# Autodesk Inventor assembly: Assembly_all
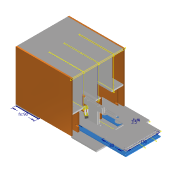
[picture p0: Inventor's stored thumbnail of the model, 180x180]
Saved by Autodesk Inventor 2020 (Build 240168000, 168)
## iProperties
Created: 2021-05-08
Part Number: Assembly_all
Document SubType Name: Assembly
Designer: Hsu Daniel
Author: Hsu Daniel
## Documents named in this file (14)
- D:\Daniel\NTU\makeNTU2021\大改\Assembly_all.iam
- D:\Daniel\NTU\makeNTU2021\大改\lr_heater_assemble.iam
- D:\Daniel\NTU\makeNTU2021\大改\mid_heater_assemble.iam
- D:\Daniel\NTU\makeNTU2021\大改\heater_top.ipt
- D:\Daniel\NTU\makeNTU2021\大改\side_wall.ipt
- D:\Daniel\NTU\makeNTU2021\大改\bottom_inner_wall.ipt
- D:\Daniel\NTU\makeNTU2021\大改\deepest_layer.ipt
- D:\Daniel\NTU\makeNTU2021\大改\Ushape_bottom.ipt
- D:\Daniel\NTU\makeNTU2021\大改\Ushape_top.ipt
- D:\Daniel\NTU\makeNTU2021\大改\Stepper 28BYJ48.ipt
- D:\Daniel\NTU\makeNTU2021\大改\motor_connect.iam
- D:\Daniel\NTU\makeNTU2021\大改\rotate_support.ipt
- D:\Daniel\NTU\makeNTU2021\大改\wire_bottom.ipt
- D:\Daniel\NTU\makeNTU2021\大改\lr_heater_assembleL.iam
## Components (18 placed, 13 different names)
1. lr_heater_assemble:1 [sub-assembly] — Flush:2, Flush:4, Mate:5, Flush:31
2. mid_heater_assemble:1 [sub-assembly] — Flush:2, Flush:4, Mate:1, Mate:2, Mate:3, Mate:9, Mate:10, Flush:28, Flush:29, Flush:32
3. heater_top:1 — Mate:1, Mate:2, Mate:3, Mate:5, Mate:6, Mate:7, Flush:7, Flush:8, Flush:27, Flush:33, Flush:34
4. side_wall:1 — Mate:6, Flush:7, Flush:18, Flush:33
5. side_wall:2 — Mate:7, Flush:8, Flush:26, Flush:34
6. bottom_inner_wall:1 — Flush:11, Flush:14, Flush:31, Mate:25, Mate:26, Mate:27, Mate:28
7. bottom_inner_wall:2 — Flush:10, Flush:11, Flush:13, Flush:14, Mate:12, Mate:24, Mate:29
8. bottom_inner_wall:3 — Flush:9, Flush:10, Flush:15, Mate:9
9. bottom_inner_wall:4 — Flush:9, Flush:13, Flush:15, Mate:10
10. deepest_layer:1 — Flush:18, Mate:12, Mate:14, Flush:26, Mate:24, Mate:25
11. Ushape_bottom:1 — Mate:14, Flush:20, Flush:21, Mate:16, Flush:32, Cylindrical:1
12. Ushape_top:1 — Flush:20, Flush:21, Mate:16, Flush:25, Mate:18, Mate:19, Mate:20, Insert:1
13. Stepper 28BYJ48:1 — Mate:17, Cylindrical:1, Insert:1, Cylindrical:2
14. motor_connect:1 [sub-assembly] — Mate:17, Cylindrical:2
15. rotate_support:1 — Flush:22, Flush:23, Flush:24, Mate:19, Mate:20
16. rotate_support:2 — Flush:22, Flush:23, Flush:24, Flush:25, Mate:18
17. lr_heater_assembleL:1 [sub-assembly] — Flush:27, Flush:28, Flush:29, Mate:29
18. wire_bottom:1 — Mate:26, Mate:27, Mate:28
## Relationships (49: Flush 25, Mate 21, CylindricalJoint 2, Insert 1)
- Flush:2: lr_heater_assemble:1 ↔ mid_heater_assemble:1
- Flush:4: lr_heater_assemble:1 ↔ mid_heater_assemble:1
- Mate:1: mid_heater_assemble:1 ↔ heater_top:1
- Mate:2: mid_heater_assemble:1 ↔ heater_top:1
- Mate:3: mid_heater_assemble:1 ↔ heater_top:1
- Mate:5: lr_heater_assemble:1 ↔ heater_top:1
- Mate:6: heater_top:1 ↔ side_wall:1
- Mate:7: heater_top:1 ↔ side_wall:2
- Flush:7: heater_top:1 ↔ side_wall:1
- Flush:8: heater_top:1 ↔ side_wall:2
- Flush:9: bottom_inner_wall:3 ↔ bottom_inner_wall:4
- Flush:10: bottom_inner_wall:2 ↔ bottom_inner_wall:3
- Flush:11: bottom_inner_wall:1 ↔ bottom_inner_wall:2
- Flush:13: bottom_inner_wall:2 ↔ bottom_inner_wall:4
- Flush:14: bottom_inner_wall:1 ↔ bottom_inner_wall:2
- Flush:15: bottom_inner_wall:3 ↔ bottom_inner_wall:4
- Mate:9: mid_heater_assemble:1 ↔ bottom_inner_wall:3
- Mate:10: mid_heater_assemble:1 ↔ bottom_inner_wall:4
- Flush:18: side_wall:1 ↔ deepest_layer:1
- Mate:12: bottom_inner_wall:2 ↔ deepest_layer:1
- Mate:14: deepest_layer:1 ↔ Ushape_bottom:1
- Flush:20: Ushape_bottom:1 ↔ Ushape_top:1
- Flush:21: Ushape_bottom:1 ↔ Ushape_top:1
- Mate:16 (16 mm): Ushape_bottom:1 ↔ Ushape_top:1
- Mate:17: Stepper 28BYJ48:1 ↔ motor_connect:1
- Flush:22: rotate_support:1 ↔ rotate_support:2
- Flush:23: rotate_support:1 ↔ rotate_support:2
- Flush:24: rotate_support:1 ↔ rotate_support:2
- Flush:25: Ushape_top:1 ↔ rotate_support:2
- Mate:18: Ushape_top:1 ↔ rotate_support:2
- Mate:19: Ushape_top:1 ↔ rotate_support:1
- Mate:20: Ushape_top:1 ↔ rotate_support:1
- Flush:26: side_wall:2 ↔ deepest_layer:1
- Flush:27: heater_top:1 ↔ lr_heater_assembleL:1
- Flush:28: mid_heater_assemble:1 ↔ lr_heater_assembleL:1
- Flush:29: mid_heater_assemble:1 ↔ lr_heater_assembleL:1
- Flush:31: lr_heater_assemble:1 ↔ bottom_inner_wall:1
- Mate:24: bottom_inner_wall:2 ↔ deepest_layer:1
- Mate:25: bottom_inner_wall:1 ↔ deepest_layer:1
- Mate:26: bottom_inner_wall:1 ↔ wire_bottom:1
- Mate:27: bottom_inner_wall:1 ↔ wire_bottom:1
- Mate:28: bottom_inner_wall:1 ↔ wire_bottom:1
- Flush:32: mid_heater_assemble:1 ↔ Ushape_bottom:1
- Mate:29: bottom_inner_wall:2 ↔ lr_heater_assembleL:1
- Cylindrical:1: Ushape_bottom:1 ↔ Stepper 28BYJ48:1
- Insert:1: Ushape_top:1 ↔ Stepper 28BYJ48:1
- Cylindrical:2: Stepper 28BYJ48:1 ↔ motor_connect:1
- Flush:33: heater_top:1 ↔ side_wall:1
- Flush:34: heater_top:1 ↔ side_wall:2
